# Autodesk Inventor assembly: Weapon Assembly
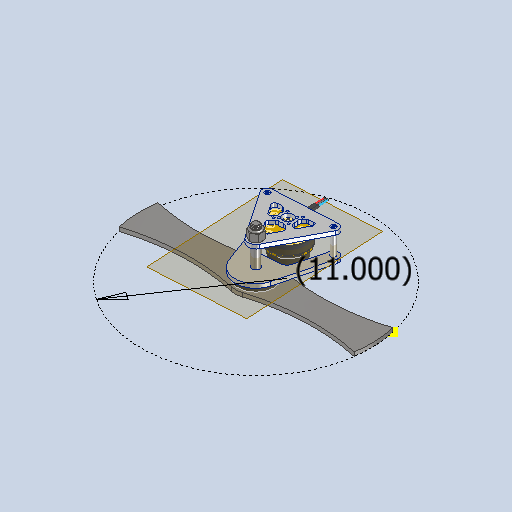
[picture p0: Inventor's stored thumbnail of the model, 512x512]
Saved by Autodesk Inventor 2023.2 (Build 272271000, 271)
## iProperties
Created: 2022-05-21
Part Number: Weapon Assembly
Document SubType Name: Assembly
Designer: Nathan Cai
Mass: 705.723 g
Surface Area: 707.55 cm^2
Volume: 130.938 cm^3
Density: 5.38974 g/cm^3
Author: Nathan Cai
## Documents named in this file (8)
- C:\Users\Nathan Cai\Documents\Inventor\0.3rd Lawette - V3.6\Horizontal Weapon Assembly (Type U)\Weapon Assembly (Horizontal U).iam
- C:\Users\Nathan Cai\Documents\Inventor\0.3rd Lawette - V3.6\Horizontal Weapon Assembly (Type U)\Weapon (Weapon-Side Pulley).iam
- C:\Users\Nathan Cai\Documents\Inventor\0.3rd Lawette - V3.6\Horizontal Weapon Assembly (Type U)\90807A139_Same-Size Thread Alloy Steel Shoulder Screw.ipt
- C:\Users\Nathan Cai\Documents\Inventor\0.3rd Lawette - V3.6\Horizontal Weapon Assembly (Type U)\90630A121_High-Strength Steel Nylon-Insert Locknut.ipt
- C:\Users\Nathan Cai\Documents\Inventor\0.3rd Lawette - V3.6\Horizontal Weapon Assembly (Type U)\Weapon (Motor-Side Pulley).iam
- C:\Users\Nathan Cai\Documents\Inventor\0.3rd Lawette - V3.6\Horizontal Weapon Assembly (Type U)\Frame (Clear Side).ipt
- C:\Users\Nathan Cai\Documents\Inventor\0.3rd Lawette - V3.6\Horizontal Weapon Assembly (Type U)\Frame (Motor Side).ipt
- C:\Users\Nathan Cai\Documents\Inventor\0.3rd Lawette - V3.6\Standoff 1.5in.ipt
## Components (8 placed, 7 different names)
1. Weapon (Weapon-Side Pulley):1 [sub-assembly] — Mate:174, Mate:191
2. 90807A139_Same-Size Thread Alloy Steel Shoulder Screw:1 — Mate:1, Mate:2, Mate:9, Mate:174
3. 90630A121_High-Strength Steel Nylon-Insert Locknut:1 — Mate:1, Mate:2, Mate:173
4. Frame (Motor Side):1 — Symmetry:1, Mate:173, Mate:187, Mate:188, Mate:189, Mate:192, Mate:193, Flush:1, Flush:2, Mate:194
5. Frame (Clear Side):1 — Mate:9, Symmetry:1, Mate:187, Mate:191
6. Weapon (Motor-Side Pulley):1 [sub-assembly] — Mate:188, Mate:189, Mate:194
7. Standoff 1.5in:1 — Mate:192, Flush:1
8. Standoff 1.5in:2 — Mate:193, Flush:2
## Relationships (17: Mate 14, Flush 2, Symmetry 1)
- Mate:1: 90807A139_Same-Size Thread Alloy Steel Shoulder Screw:1 ↔ 90630A121_High-Strength Steel Nylon-Insert Locknut:1
- Mate:2 (47.625 mm): 90807A139_Same-Size Thread Alloy Steel Shoulder Screw:1 ↔ 90630A121_High-Strength Steel Nylon-Insert Locknut:1
- [Mate]: 90807A139_Same-Size Thread Alloy Steel Shoulder Screw:1 ↔ Frame (Motor Side):1
- Mate:9: 90807A139_Same-Size Thread Alloy Steel Shoulder Screw:1 ↔ Frame (Clear Side):1
- [Mate]: Frame (Motor Side):1 ↔ Frame (Clear Side):1
- Symmetry:1: Frame (Motor Side):1 ↔ Frame (Clear Side):1
- Mate:173: 90630A121_High-Strength Steel Nylon-Insert Locknut:1 ↔ Frame (Motor Side):1
- Mate:174: Weapon (Weapon-Side Pulley):1 ↔ 90807A139_Same-Size Thread Alloy Steel Shoulder Screw:1
- Mate:187 (25.4 mm): Frame (Motor Side):1 ↔ Frame (Clear Side):1
- Mate:188: Frame (Motor Side):1 ↔ Weapon (Motor-Side Pulley):1
- Mate:189: Frame (Motor Side):1 ↔ Weapon (Motor-Side Pulley):1
- Mate:191: Weapon (Weapon-Side Pulley):1 ↔ Frame (Clear Side):1
- Mate:192: Frame (Motor Side):1 ↔ Standoff 1.5in:1
- Mate:193: Frame (Motor Side):1 ↔ Standoff 1.5in:2
- Flush:1: Frame (Motor Side):1 ↔ Standoff 1.5in:1
- Flush:2: Frame (Motor Side):1 ↔ Standoff 1.5in:2
- Mate:194: Frame (Motor Side):1 ↔ Weapon (Motor-Side Pulley):1
